# Autodesk Inventor assembly: support_engine
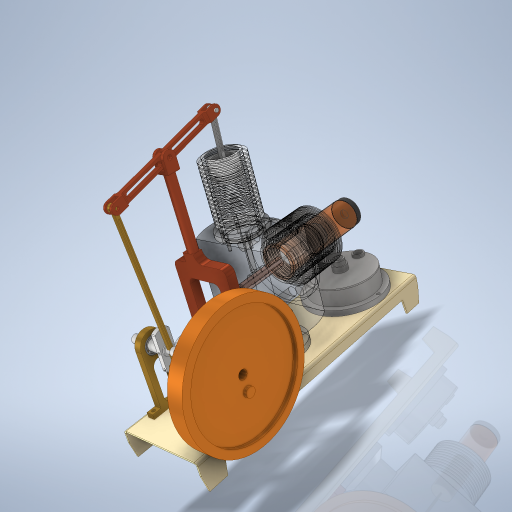
[picture p0: Inventor's stored thumbnail of the model, 512x512]
Saved by Autodesk Inventor 2024.2 (Build 282272000, 272)
## iProperties
Created: 2024-05-04
Part Number: support_engine
Document SubType Name: Assembly
Designer: Fabri
Author: Fabri
## Documents named in this file (28)
- C:\Users\Fabri\Documents\Inventor\stirlingEngine\support_engine.iam
- C:\Users\Fabri\Documents\Inventor\stirlingEngine\9.ipt
- C:\Users\Fabri\Documents\Inventor\stirlingEngine\2.ipt
- C:\Users\Fabri\Documents\Inventor\stirlingEngine\1.ipt
- C:\Users\Fabri\Documents\Inventor\stirlingEngine\3.ipt
- C:\Users\Fabri\Documents\Inventor\stirlingEngine\6.ipt
- C:\Users\Fabri\Documents\Inventor\stirlingEngine\4.ipt
- C:\Users\Fabri\Documents\Inventor\stirlingEngine\5.ipt
- C:\Users\Fabri\Documents\Inventor\stirlingEngine\DIN 625 SKF - SKF 62_28.ipt
- C:\Users\Fabri\Documents\Inventor\stirlingEngine\10.ipt
- C:\Users\Fabri\Documents\Inventor\stirlingEngine\11.ipt
- C:\Users\Fabri\Documents\Inventor\stirlingEngine\12.ipt
- C:\Users\Fabri\Documents\Inventor\stirlingEngine\14.ipt
- C:\Users\Fabri\Documents\Inventor\stirlingEngine\15.ipt
- C:\Users\Fabri\Documents\Inventor\stirlingEngine\13.ipt
- C:\Users\Fabri\Documents\Inventor\stirlingEngine\16.ipt
- C:\Users\Fabri\Documents\Inventor\stirlingEngine\kolben.ipt
- C:\Users\Fabri\Documents\Inventor\stirlingEngine\kolbenzapfen.ipt
- C:\Users\Fabri\Documents\Inventor\stirlingEngine\pleuel_third.ipt
- C:\Users\Fabri\Documents\Inventor\stirlingEngine\pleuel_rad.ipt
- C:\Users\Fabri\Documents\Inventor\stirlingEngine\cylinder_assembly.iam
- C:\Users\Fabri\Documents\Inventor\stirlingEngine\19.ipt
- C:\Users\Fabri\Documents\Inventor\stirlingEngine\wheel_support.ipt
- C:\Users\Fabri\Documents\Inventor\stirlingEngine\pleuel_rad_2.ipt
- C:\Users\Fabri\Documents\Inventor\stirlingEngine\rad.ipt
- C:\Users\Fabri\Documents\Inventor\stirlingEngine\connection_6_1.iam
- C:\Users\Fabri\Documents\Inventor\stirlingEngine\bolt.ipt
- C:\Users\Fabri\Documents\Inventor\stirlingEngine\vernindung.ipt
## Components (32 placed, 27 different names)
1. 9:1 — Passend:1, Einfügen:1, Passend:3, Einfügen:3, Passend:6, Einfügen:6, Passend:8, Einfügen:8, Passend:11, Einfügen:11
2. 2:1 — Passend:1, Einfügen:1, Passend:4, Einfügen:4, Winkel:1, Winkel:5
3. 1:1 — Passend:8, Einfügen:8, Einfügen:9
4. 1:2 — Passend:3, Einfügen:3, Einfügen:10
5. 3:1 — Passend:4, Einfügen:4, Passend:5, Einfügen:5
6. 6:1 — Passend:5, Einfügen:5, Winkel:1, Einfügen:16
7. 4:1 — Passend:6, Einfügen:6, Passend:7, Einfügen:7
8. 5:1 — Passend:7, Einfügen:7, Winkel:2
9. DIN 625 SKF - SKF 62_28:1 — Einfügen:9
10. DIN 625 SKF - SKF 62_28:2 — Einfügen:10, Einfügen:46
11. 10:1 — Passend:11, Einfügen:11, Winkel:5, Passend:18, Einfügen:18, Einfügen:41, Einfügen:42
12. 11:1 — Einfügen:53
13. 12:1 — Einfügen:53
14. 15:1 — Einfügen:41, Zylindrisch:6
15. 13:1 — Einfügen:42
16. 16:1 — Einfügen:16, Einfügen:37, Einfügen:39, Passend:28
17. kolben:1 — Zylindrisch:4, Zylindrisch:5
18. kolbenzapfen:1 — Zylindrisch:5, Einfügen:38
19. pleuel_third:1 — Einfügen:38, Einfügen:39
20. 14:1 — Passend:18, Einfügen:18, Zylindrisch:4
21. pleuel_rad:1 — Passend:27, Passend:28, Einfügen:51
22. cylinder_assembly:1 [sub-assembly] — Zylindrisch:6, Passend:30, Einfügen:52
23. wheel_support:1 — Passend:20, Fluchtend:1, Einfügen:49
24. 19:2 — Winkel:9, Einfügen:46, Einfügen:47, Einfügen:49, Passend:23, Passend:25
25. wheel_support:2 — Passend:21, Fluchtend:2, Einfügen:50
26. 19:4
27. pleuel_rad_2:1 — Passend:29, Passend:30, Einfügen:52
28. rad:1 — Winkel:9, Einfügen:47, Passend:22, Winkel:11, Passend:25, Passend:26, Main_motion, Winkel:13, Winkel:14
29. connection_6_1:1 [sub-assembly] — Passend:20, Fluchtend:1, Passend:21, Fluchtend:2, Winkel:13, Passend:27, Einfügen:51, Passend:29
30. bolt:1 — Einfügen:37
31. 19:5 — Passend:22, Winkel:11, Einfügen:50, Passend:26
32. vernindung:1 — Passend:23, Winkel:14
## Relationships (56: Insert 24, Mate 19, Angle 8, CylindricalJoint 3, Flush 2)
- Passend:1 [Mate]: 9:1 ↔ 2:1
- Einfügen:1 [Insert]: 9:1 ↔ 2:1
- Passend:3 [Mate]: 9:1 ↔ 1:2
- Einfügen:3 [Insert]: 9:1 ↔ 1:2
- Passend:4 [Mate]: 2:1 ↔ 3:1
- Einfügen:4 [Insert]: 2:1 ↔ 3:1
- Passend:5 [Mate]: 3:1 ↔ 6:1
- Einfügen:5 [Insert] (-24.5 mm): 3:1 ↔ 6:1
- Winkel:1 [Angle] (90 deg): 2:1 ↔ 6:1
- Passend:6 [Mate]: 9:1 ↔ 4:1
- Einfügen:6 [Insert]: 9:1 ↔ 4:1
- Passend:7 [Mate]: 4:1 ↔ 5:1
- Einfügen:7 [Insert] (-4.8 mm): 4:1 ↔ 5:1
- Winkel:2 [Angle] (180 deg): 5:1
- Passend:8 [Mate]: 9:1 ↔ 1:1
- Einfügen:8 [Insert]: 9:1 ↔ 1:1
- Einfügen:9 [Insert] (-18 mm): 1:1 ↔ DIN 625 SKF - SKF 62_28:1
- Einfügen:10 [Insert] (-18 mm): 1:2 ↔ DIN 625 SKF - SKF 62_28:2
- Passend:11 [Mate]: 9:1 ↔ 10:1
- Einfügen:11 [Insert]: 9:1 ↔ 10:1
- Einfügen:16 [Insert] (2 mm): 6:1 ↔ 16:1
- Winkel:5 [Angle] (180 deg): 2:1 ↔ 10:1
- Passend:18 [Mate]: 10:1 ↔ 14:1
- Einfügen:18 [Insert] (-9 mm): 10:1 ↔ 14:1
- Einfügen:37 [Insert] (-36 mm): 16:1 ↔ bolt:1
- Zylindrisch:4 [CylindricalJoint]: kolben:1 ↔ 14:1
- Zylindrisch:5 [CylindricalJoint]: kolben:1 ↔ kolbenzapfen:1
- Einfügen:38 [Insert] (-58 mm): kolbenzapfen:1 ↔ pleuel_third:1
- Einfügen:39 [Insert] (2 mm): 16:1 ↔ pleuel_third:1
- Einfügen:41 [Insert] (-160 mm): 10:1 ↔ 15:1
- Einfügen:42 [Insert] (168 mm): 10:1 ↔ 13:1
- Zylindrisch:6 [CylindricalJoint]: 15:1 ↔ cylinder_assembly:1
- Winkel:9 [Angle] (90 deg): 19:2 ↔ rad:1
- Einfügen:46 [Insert]: DIN 625 SKF - SKF 62_28:2 ↔ 19:2
- Einfügen:47 [Insert] (-10 mm): 19:2 ↔ rad:1
- Passend:20 [Mate]: wheel_support:1 ↔ connection_6_1:1
- Fluchtend:1 [Flush]: wheel_support:1 ↔ connection_6_1:1
- Passend:21 [Mate]: wheel_support:2 ↔ connection_6_1:1
- Fluchtend:2 [Flush]: wheel_support:2 ↔ connection_6_1:1
- Einfügen:49 [Insert] (-20 mm): wheel_support:1 ↔ 19:2
- Passend:22 [Mate]: rad:1 ↔ 19:5
- Winkel:11 [Angle] (90 deg): rad:1 ↔ 19:5
- Einfügen:50 [Insert] (-20 mm): wheel_support:2 ↔ 19:5
- Passend:23 [Mate]: 19:2 ↔ vernindung:1
- Passend:25 [Mate]: 19:2 ↔ rad:1
- Passend:26 [Mate]: rad:1 ↔ 19:5
- Main_motion [Angle] (0 deg): rad:1
- Winkel:13 [Angle] (270 deg): rad:1 ↔ connection_6_1:1
- Winkel:14 [Angle] (0 deg): rad:1 ↔ vernindung:1
- Passend:27 [Mate]: pleuel_rad:1 ↔ connection_6_1:1
- Passend:28 [Mate]: 16:1 ↔ pleuel_rad:1
- Einfügen:51 [Insert] (-42 mm): pleuel_rad:1 ↔ connection_6_1:1
- Passend:29 [Mate]: pleuel_rad_2:1 ↔ connection_6_1:1
- Passend:30 [Mate]: cylinder_assembly:1 ↔ pleuel_rad_2:1
- Einfügen:52 [Insert]: cylinder_assembly:1 ↔ pleuel_rad_2:1
- Einfügen:53 [Insert]: 11:1 ↔ 12:1
